# Autodesk Inventor assembly: Assembly1
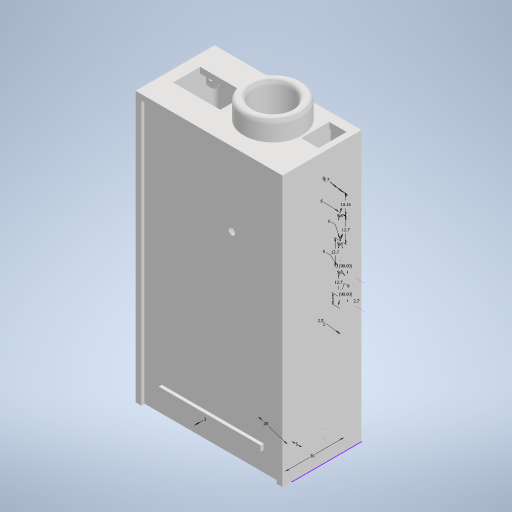
[picture p0: Inventor's stored thumbnail of the model, 512x512]
Saved by Autodesk Inventor 2023 (Build 270158000, 158)
## iProperties
Created: 2024-03-30
Part Number: Assembly1
Document SubType Name: Assembly
Designer: lykou
Author: lykou
## Documents named in this file (4)
- D:\My Drive\Documents\Projects\pico_chrono\Open-Source-Chronograph\CAD\Assembly1.iam
- D:\My Drive\Documents\Projects\pico_chrono\Open-Source-Chronograph\CAD\MainBody.ipt
- D:\My Drive\Documents\Projects\pico_chrono\Open-Source-Chronograph\CAD\Button.ipt
- D:\My Drive\Documents\Projects\pico_chrono\Open-Source-Chronograph\CAD\Lid.ipt
## Components (5 placed, 3 different names)
1. MainBody:1 — Mate:1, Mate:2, Mate:3, Mate:4, Mate:5, Mate:6, Mate:7, Mate:8, Mate:9, Mate:10
2. Button:1 — Mate:3, Mate:4
3. Button:2 — Mate:5, Mate:6
4. Button:3 — Mate:1, Mate:2
5. Lid:1 — Mate:7, Mate:8, Mate:9, Mate:10
## Relationships (10: Mate 10)
- Mate:1: MainBody:1 ↔ Button:3
- Mate:2: MainBody:1 ↔ Button:3
- Mate:3: MainBody:1 ↔ Button:1
- Mate:4: MainBody:1 ↔ Button:1
- Mate:5: MainBody:1 ↔ Button:2
- Mate:6: MainBody:1 ↔ Button:2
- Mate:7: MainBody:1 ↔ Lid:1
- Mate:8: MainBody:1 ↔ Lid:1
- Mate:9: MainBody:1 ↔ Lid:1
- Mate:10: MainBody:1 ↔ Lid:1
